# Autodesk Inventor assembly: Test Assembly
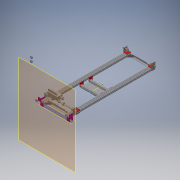
[picture p0: Inventor's stored thumbnail of the model, 180x180]
Saved by Autodesk Inventor 2016 SP2 (Build 200236200, 236)
## iProperties
Created: 2018-01-27
Part Number: Test Assembly
Document SubType Name: Assembly
Designer: CAD
Author: CAD
## Documents named in this file (20)
- C:\Users\CAD\Documents\GitHub\FIRST-ROBOTICS-2018-5436-CAD\Robot\Elevator\Test Assembly.iam
- C:\Users\CAD\Documents\GitHub\FIRST-ROBOTICS-2018-5436-CAD\Robot\Elevator\48 in 80-20 extrusion.ipt
- C:\Users\CAD\Documents\GitHub\FIRST-ROBOTICS-2018-5436-CAD\Robot\Elevator\80-20 extrusion rail.ipt
- C:\Users\CAD\Documents\GitHub\FIRST-ROBOTICS-2018-5436-CAD\Robot\Elevator\Bottom Elevator Bracket.ipt
- C:\Users\CAD\Documents\GitHub\FIRST-ROBOTICS-2018-5436-CAD\Robot\Elevator\10.75 in 80-20 extrusion.ipt
- C:\Users\CAD\Documents\GitHub\FIRST-ROBOTICS-2018-5436-CAD\Robot\Elevator\Triangle Bracket.ipt
- C:\Users\CAD\Documents\GitHub\FIRST-ROBOTICS-2018-5436-CAD\Robot\Elevator\11.25 in L.ipt
- C:\Users\CAD\Documents\GitHub\FIRST-ROBOTICS-2018-5436-CAD\Robot\Elevator\Upper Bracket of Elevator.ipt
- C:\Users\CAD\Documents\GitHub\FIRST-ROBOTICS-2018-5436-CAD\Robot\Elevator\hex axle for elevator.ipt
- C:\Users\CAD\Documents\GitHub\FIRST-ROBOTICS-2018-5436-CAD\Robot\Climbing Pieces\drive motor + trasmission pieces\Collar.ipt
- C:\Users\CAD\Documents\GitHub\FIRST-ROBOTICS-2018-5436-CAD\Robot\Elevator\Back Plate.ipt
- C:\Users\CAD\Documents\GitHub\FIRST-ROBOTICS-2018-5436-CAD\Robot\Elevator\Bearing.ipt
- C:\Users\CAD\Documents\GitHub\FIRST-ROBOTICS-2018-5436-CAD\Robot\Elevator\rope connection to cart.ipt
- C:\Users\CAD\Documents\GitHub\FIRST-ROBOTICS-2018-5436-CAD\Robot\Elevator\small hex axle top elevator.ipt
- C:\Users\CAD\Documents\GitHub\FIRST-ROBOTICS-2018-5436-CAD\Robot\Elevator\Bottom Elevator Bracket Square.ipt
- C:\Users\CAD\Documents\Vault\climbing\Climbing sprocket.ipt
- C:\Users\CAD\Documents\GitHub\FIRST-ROBOTICS-2018-5436-CAD\Robot\Elevator\Bag elevator Motor.ipt
- C:\Users\CAD\Documents\GitHub\FIRST-ROBOTICS-2018-5436-CAD\Robot\Elevator\Ls in motor tensioner.ipt
- C:\Users\CAD\Documents\GitHub\FIRST-ROBOTICS-2018-5436-CAD\Robot\Elevator\Motor Tension Block Mount.ipt
- C:\Users\CAD\Documents\GitHub\FIRST-ROBOTICS-2018-5436-CAD\Robot\Elevator\.5 in spacer.ipt
## Components (60 placed, 19 different names)
1. 48 in 80-20 extrusion:1 — Flush:1, Flush:3, Flush:5, Mate:16, Flush:12, Mate:26, Mate:27, Mate:70, Mate:71, Flush:27, Mate:83, Mate:84, Mate:98
2. 48 in 80-20 extrusion:2 — Flush:1, Mate:2, Mate:3, Mate:4, Mate:5, Flush:2, Mate:8, Mate:9, Mate:10, Mate:11, Flush:8, Flush:11, Mate:34, Mate:35, Mate:44, Mate:45, Mate:50, Mate:51, Mate:52, Mate:61, Mate:62, Flush:21
3. 48 in 80-20 extrusion:3 — Flush:5, Flush:6, Mate:19, Flush:11, Flush:13, Flush:14, Mate:39, Mate:40, Mate:46, Mate:47, Mate:53, Mate:54, Mate:58, Mate:59, Mate:60, Mate:67
4. 48 in 80-20 extrusion:4 — Flush:6, Mate:17, Mate:18, Mate:20, Mate:21, Flush:9, Flush:10, Flush:12, Mate:22, Mate:23, Mate:24, Mate:25, Mate:28, Mate:29, Flush:16, Mate:68, Mate:69, Mate:81, Mate:82, Flush:29, Mate:96
5. 80-20 extrusion rail:1 — Mate:2, Mate:3, Flush:2, Mate:6
6. 80-20 extrusion rail:2 — Mate:8, Mate:9, Flush:7, Mate:16
7. 80-20 extrusion rail:3 — Mate:10, Mate:11, Flush:8
8. 80-20 extrusion rail:4 — Mate:4, Mate:5, Flush:3, Mate:6, Flush:7
9. 80-20 extrusion rail:5 — Mate:17, Mate:18, Mate:19, Flush:9
10. 80-20 extrusion rail:8 — Mate:20, Mate:21, Flush:10
11. 80-20 extrusion rail:9 — Mate:24, Mate:25, Flush:14
12. 80-20 extrusion rail:10 — Mate:22, Mate:23, Flush:13
13. Bottom Elevator Bracket:1 — Mate:26, Mate:27, Flush:15, Angle:3, Flush:34, Mate:99
14. Bottom Elevator Bracket:2 — Mate:28, Mate:29, Flush:15, Flush:16, Mate:38, Flush:33, Mate:97, Flush:119
15. 80-20 extrusion rail:11 — Angle:2, Mate:39, Mate:40, Flush:17, Mate:41, Angle:4
16. 80-20 extrusion rail:12 — Mate:34, Mate:35, Angle:2, Flush:17, Mate:42, Mate:43, Mate:65
17. 10.75 in 80-20 extrusion:1 — Mate:41, Mate:42, Mate:43, Angle:4, Mate:66
18. Triangle Bracket:1 — Mate:44, Mate:45, Flush:18
19. Triangle Bracket:2 — Mate:46, Mate:47, Flush:18, Mate:48, Mate:49, Mate:67
20. 11.25 in L:1 — Mate:48, Mate:49, Mate:50
21. Triangle Bracket:3 — Mate:51, Mate:52, Mate:57, Flush:21
22. Triangle Bracket:4 — Mate:53, Mate:54, Mate:55, Mate:56
23. 11.25 in L:2 — Mate:55, Mate:56, Mate:57, Mate:58, Mate:65
24. 10.75 in 80-20 extrusion:2 — Mate:63, Mate:64, Angle:5, Mate:66, Mate:79, Flush:28, Mate:94, Mate:95
25. 80-20 extrusion rail:13 — Mate:59, Mate:60, Flush:19, Mate:63, Mate:80
26. 80-20 extrusion rail:14 — Mate:61, Mate:62, Flush:19, Mate:64, Angle:5
27. Upper Bracket of Elevator:1 — Mate:70, Mate:71, Flush:27, Insert:1
28. Upper Bracket of Elevator:2 — Mate:68, Mate:69, Mate:77, Flush:30, Insert:3, Mate:100
29. Collar:1 — Mate:73, Mate:74, Mate:77, Mate:87
30. Collar:2 — Mate:75, Mate:76, Mate:88
31. hex axle for elevator:1 — Mate:73, Mate:74, Mate:75, Mate:76, Flush:31, Mate:89, Mate:90, Mate:91, Mate:92, Mate:101, Mate:102, Mate:111, Mate:130, Mate:133, Mate:136
32. Back Plate:1 — Mate:79, Flush:28, Mate:80, Flush:32
33. Upper Bracket of Elevator:3 — Mate:83, Mate:84, Flush:30, Mate:85, Mate:86
34. Upper Bracket of Elevator:4 — Mate:81, Mate:82, Flush:29, Insert:2
35. Bearing:1 — Mate:85, Mate:86, Mate:87, Flush:31
36. Bearing:2 — Insert:2, Mate:109, Mate:138
37. Bearing:3 — Insert:3, Mate:88
38. Bearing:4 — Insert:1, Mate:106, Mate:137
39. rope connection to cart:1 — Mate:94, Mate:95, Flush:32
40. Collar:3 — Mate:89, Mate:90, Mate:93, Mate:103
41. Collar:4 — Mate:91, Mate:92, Mate:93
42. small hex axle top elevator:1 — Mate:108, Mate:135, Flush:128
43. small hex axle top elevator:2 — Mate:105, Mate:132, Flush:127
44. Bottom Elevator Bracket Square:1 — Flush:33, Mate:96, Mate:97, Mate:100
45. Bottom Elevator Bracket Square:3 — Mate:98, Flush:34, Mate:99
46. Climbing sprocket:1 — Mate:101, Mate:102, Mate:103, Mate:128
47. Climbing sprocket:2 — Mate:108, Mate:109, Mate:135, Flush:126, Mate:138, Flush:128
48. Climbing sprocket:3
49. Climbing sprocket:4 — Mate:130, Flush:126, Mate:136
50. Climbing sprocket:5 — Mate:105, Mate:106, Flush:35, Mate:132, Mate:137, Flush:127
51. Climbing sprocket:6 — Mate:111, Flush:35, Mate:133
52. Climbing sprocket:7 — Mate:120, Mate:121, Mate:122, Mate:123, Mate:124, Mate:128
53. Bag elevator Motor:1 — Mate:113, Flush:38, Flush:39, Mate:120, Mate:121, Mate:122, Mate:125, Mate:126
54. Ls in motor tensioner:1 — Mate:117, Flush:40, Flush:41, Flush:120
55. Ls in motor tensioner:2 — Mate:114, Mate:115, Mate:116, Mate:117, Flush:40, Flush:41
56. Motor Tension Block Mount:1 — Mate:113, Flush:38, Flush:39, Mate:114, Mate:115, Mate:116
57. .5 in spacer:1 — Mate:123, Mate:124, Mate:127
58. Collar:5 — Mate:125, Mate:126, Mate:127
59. Collar:6
60. Collar:7
## Relationships (159: Mate 115, Flush 37, Angle 4, Insert 3)
- Flush:1: 48 in 80-20 extrusion:1 ↔ 48 in 80-20 extrusion:2
- Mate:2: 48 in 80-20 extrusion:2 ↔ 80-20 extrusion rail:1
- Mate:3: 48 in 80-20 extrusion:2 ↔ 80-20 extrusion rail:1
- Mate:4: 48 in 80-20 extrusion:2 ↔ 80-20 extrusion rail:4
- Mate:5: 48 in 80-20 extrusion:2 ↔ 80-20 extrusion rail:4
- Flush:2 (101.6 mm): 48 in 80-20 extrusion:2 ↔ 80-20 extrusion rail:1
- Flush:3: 48 in 80-20 extrusion:1 ↔ 80-20 extrusion rail:4
- Mate:6 (136.7282 mm): 80-20 extrusion rail:1 ↔ 80-20 extrusion rail:4
- Flush:5: 48 in 80-20 extrusion:1 ↔ 48 in 80-20 extrusion:3
- Flush:6: 48 in 80-20 extrusion:3 ↔ 48 in 80-20 extrusion:4
- Mate:8: 48 in 80-20 extrusion:2 ↔ 80-20 extrusion rail:2
- Mate:9: 48 in 80-20 extrusion:2 ↔ 80-20 extrusion rail:2
- Flush:7: 80-20 extrusion rail:2 ↔ 80-20 extrusion rail:4
- Mate:10: 48 in 80-20 extrusion:2 ↔ 80-20 extrusion rail:3
- Mate:11: 48 in 80-20 extrusion:2 ↔ 80-20 extrusion rail:3
- Flush:8 (101.6 mm): 48 in 80-20 extrusion:2 ↔ 80-20 extrusion rail:3
- Mate:16: 48 in 80-20 extrusion:1 ↔ 80-20 extrusion rail:2
- Mate:17: 48 in 80-20 extrusion:4 ↔ 80-20 extrusion rail:5
- Mate:18: 48 in 80-20 extrusion:4 ↔ 80-20 extrusion rail:5
- Mate:19: 48 in 80-20 extrusion:3 ↔ 80-20 extrusion rail:5
- Mate:20: 48 in 80-20 extrusion:4 ↔ 80-20 extrusion rail:8
- Mate:21: 48 in 80-20 extrusion:4 ↔ 80-20 extrusion rail:8
- Flush:9: 48 in 80-20 extrusion:4 ↔ 80-20 extrusion rail:5
- Flush:10: 48 in 80-20 extrusion:4 ↔ 80-20 extrusion rail:8
- Flush:11: 48 in 80-20 extrusion:2 ↔ 48 in 80-20 extrusion:3
- Flush:12: 48 in 80-20 extrusion:1 ↔ 48 in 80-20 extrusion:4
- Mate:22: 48 in 80-20 extrusion:4 ↔ 80-20 extrusion rail:10
- Mate:23: 48 in 80-20 extrusion:4 ↔ 80-20 extrusion rail:10
- Flush:13 (101.6 mm): 48 in 80-20 extrusion:3 ↔ 80-20 extrusion rail:10
- Mate:24: 48 in 80-20 extrusion:4 ↔ 80-20 extrusion rail:9
- Mate:25: 48 in 80-20 extrusion:4 ↔ 80-20 extrusion rail:9
- Flush:14 (-101.6 mm): 48 in 80-20 extrusion:3 ↔ 80-20 extrusion rail:9
- Mate:26: 48 in 80-20 extrusion:1 ↔ Bottom Elevator Bracket:1
- Mate:27: 48 in 80-20 extrusion:1 ↔ Bottom Elevator Bracket:1
- Mate:28: 48 in 80-20 extrusion:4 ↔ Bottom Elevator Bracket:2
- Mate:29: 48 in 80-20 extrusion:4 ↔ Bottom Elevator Bracket:2
- Flush:15: Bottom Elevator Bracket:1 ↔ Bottom Elevator Bracket:2
- Flush:16: 48 in 80-20 extrusion:4 ↔ Bottom Elevator Bracket:2
- Mate:34: 48 in 80-20 extrusion:2 ↔ 80-20 extrusion rail:12
- Mate:35: 48 in 80-20 extrusion:2 ↔ 80-20 extrusion rail:12
- Angle:2 (0 deg): 80-20 extrusion rail:11 ↔ 80-20 extrusion rail:12
- Mate:38: Bottom Elevator Bracket:2
- Angle:3 (0 deg): Bottom Elevator Bracket:1
- Mate:39: 48 in 80-20 extrusion:3 ↔ 80-20 extrusion rail:11
- Mate:40: 48 in 80-20 extrusion:3 ↔ 80-20 extrusion rail:11
- Flush:17: 80-20 extrusion rail:11 ↔ 80-20 extrusion rail:12
- Mate:41: 80-20 extrusion rail:11 ↔ 10.75 in 80-20 extrusion:1
- Mate:42: 80-20 extrusion rail:12 ↔ 10.75 in 80-20 extrusion:1
- Mate:43: 80-20 extrusion rail:12 ↔ 10.75 in 80-20 extrusion:1
- Angle:4 (0 deg): 80-20 extrusion rail:11 ↔ 10.75 in 80-20 extrusion:1
- Mate:44: 48 in 80-20 extrusion:2 ↔ Triangle Bracket:1
- Mate:45: 48 in 80-20 extrusion:2 ↔ Triangle Bracket:1
- Mate:46: 48 in 80-20 extrusion:3 ↔ Triangle Bracket:2
- Mate:47: 48 in 80-20 extrusion:3 ↔ Triangle Bracket:2
- Flush:18: Triangle Bracket:1 ↔ Triangle Bracket:2
- Mate:48: Triangle Bracket:2 ↔ 11.25 in L:1
- Mate:49: Triangle Bracket:2 ↔ 11.25 in L:1
- Mate:50 (1.27 mm): 48 in 80-20 extrusion:2 ↔ 11.25 in L:1
- Mate:51: 48 in 80-20 extrusion:2 ↔ Triangle Bracket:3
- Mate:52: 48 in 80-20 extrusion:2 ↔ Triangle Bracket:3
- Mate:53: 48 in 80-20 extrusion:3 ↔ Triangle Bracket:4
- Mate:54: 48 in 80-20 extrusion:3 ↔ Triangle Bracket:4
- Mate:55: Triangle Bracket:4 ↔ 11.25 in L:2
- Mate:56: Triangle Bracket:4 ↔ 11.25 in L:2
- Mate:57: Triangle Bracket:3 ↔ 11.25 in L:2
- Mate:58 (1.27 mm): 48 in 80-20 extrusion:3 ↔ 11.25 in L:2
- Mate:59: 48 in 80-20 extrusion:3 ↔ 80-20 extrusion rail:13
- Mate:60: 48 in 80-20 extrusion:3 ↔ 80-20 extrusion rail:13
- Mate:61: 48 in 80-20 extrusion:2 ↔ 80-20 extrusion rail:14
- Mate:62: 48 in 80-20 extrusion:2 ↔ 80-20 extrusion rail:14
- Flush:19: 80-20 extrusion rail:13 ↔ 80-20 extrusion rail:14
- Mate:63: 10.75 in 80-20 extrusion:2 ↔ 80-20 extrusion rail:13
- Mate:64: 10.75 in 80-20 extrusion:2 ↔ 80-20 extrusion rail:14
- Flush:21: 48 in 80-20 extrusion:2 ↔ Triangle Bracket:3
- Mate:65: 80-20 extrusion rail:12 ↔ 11.25 in L:2
- Angle:5 (0 deg): 10.75 in 80-20 extrusion:2 ↔ 80-20 extrusion rail:14
- Mate:66 (101.6 mm): 10.75 in 80-20 extrusion:1 ↔ 10.75 in 80-20 extrusion:2
- Mate:67 (-60.325 mm): 48 in 80-20 extrusion:3 ↔ Triangle Bracket:2
- Mate:68: 48 in 80-20 extrusion:4 ↔ Upper Bracket of Elevator:2
- Mate:69: 48 in 80-20 extrusion:4 ↔ Upper Bracket of Elevator:2
- Mate:70: 48 in 80-20 extrusion:1 ↔ Upper Bracket of Elevator:1
- Mate:71: 48 in 80-20 extrusion:1 ↔ Upper Bracket of Elevator:1
- Mate:73: Collar:1 ↔ hex axle for elevator:1
- Mate:74: Collar:1 ↔ hex axle for elevator:1
- Mate:75: Collar:2 ↔ hex axle for elevator:1
- Mate:76: Collar:2 ↔ hex axle for elevator:1
- Mate:77: Upper Bracket of Elevator:2 ↔ Collar:1
- Flush:27: 48 in 80-20 extrusion:1 ↔ Upper Bracket of Elevator:1
- Mate:79: 10.75 in 80-20 extrusion:2 ↔ Back Plate:1
- Flush:28: 10.75 in 80-20 extrusion:2 ↔ Back Plate:1
- Mate:80: 80-20 extrusion rail:13 ↔ Back Plate:1
- Mate:81: 48 in 80-20 extrusion:4 ↔ Upper Bracket of Elevator:4
- Mate:82: 48 in 80-20 extrusion:4 ↔ Upper Bracket of Elevator:4
- Flush:29: 48 in 80-20 extrusion:4 ↔ Upper Bracket of Elevator:4
- Mate:83: 48 in 80-20 extrusion:1 ↔ Upper Bracket of Elevator:3
- Mate:84: 48 in 80-20 extrusion:1 ↔ Upper Bracket of Elevator:3
- Flush:30: Upper Bracket of Elevator:2 ↔ Upper Bracket of Elevator:3
- Mate:85: Upper Bracket of Elevator:3 ↔ Bearing:1
- Mate:86: Upper Bracket of Elevator:3 ↔ Bearing:1
- Insert:1: Upper Bracket of Elevator:1 ↔ Bearing:4
- Insert:2: Upper Bracket of Elevator:4 ↔ Bearing:2
- Insert:3: Upper Bracket of Elevator:2 ↔ Bearing:3
- Mate:87: Collar:1 ↔ Bearing:1
- Mate:88: Collar:2 ↔ Bearing:3
- Flush:31 (-23.5585 mm): hex axle for elevator:1 ↔ Bearing:1
- Mate:89: hex axle for elevator:1 ↔ Collar:3
- Mate:90: hex axle for elevator:1 ↔ Collar:3
- Mate:91: hex axle for elevator:1 ↔ Collar:4
- Mate:92: hex axle for elevator:1 ↔ Collar:4
- Mate:93 (50.8 mm): Collar:3 ↔ Collar:4
- Mate:94: 10.75 in 80-20 extrusion:2 ↔ rope connection to cart:1
- Mate:95: 10.75 in 80-20 extrusion:2 ↔ rope connection to cart:1
- Flush:32: Back Plate:1 ↔ rope connection to cart:1
- Flush:33: Bottom Elevator Bracket:2 ↔ Bottom Elevator Bracket Square:1
- Mate:96: 48 in 80-20 extrusion:4 ↔ Bottom Elevator Bracket Square:1
- Mate:97: Bottom Elevator Bracket:2 ↔ Bottom Elevator Bracket Square:1
- Mate:98: 48 in 80-20 extrusion:1 ↔ Bottom Elevator Bracket Square:3
- Flush:34: Bottom Elevator Bracket:1 ↔ Bottom Elevator Bracket Square:3
- Mate:99: Bottom Elevator Bracket:1 ↔ Bottom Elevator Bracket Square:3
- Mate:100: Upper Bracket of Elevator:2 ↔ Bottom Elevator Bracket Square:1
- Mate:101: hex axle for elevator:1 ↔ Climbing sprocket:1
- Mate:102: hex axle for elevator:1 ↔ Climbing sprocket:1
- Mate:103: Collar:3 ↔ Climbing sprocket:1
- Mate:105: small hex axle top elevator:2 ↔ Climbing sprocket:5
- Mate:106: Bearing:4 ↔ Climbing sprocket:5
- Mate:108: small hex axle top elevator:1 ↔ Climbing sprocket:2
- Mate:109: Bearing:2 ↔ Climbing sprocket:2
- Mate:111: hex axle for elevator:1 ↔ Climbing sprocket:6
- Flush:35: Climbing sprocket:5 ↔ Climbing sprocket:6
- Mate:113: Bag elevator Motor:1 ↔ Motor Tension Block Mount:1
- Flush:38: Bag elevator Motor:1 ↔ Motor Tension Block Mount:1
- Flush:39 (3.175 mm): Bag elevator Motor:1 ↔ Motor Tension Block Mount:1
- Mate:114: Ls in motor tensioner:2 ↔ Motor Tension Block Mount:1
- Mate:115: Ls in motor tensioner:2 ↔ Motor Tension Block Mount:1
- Mate:116: Ls in motor tensioner:2 ↔ Motor Tension Block Mount:1
- Mate:117 (114.3 mm): Ls in motor tensioner:1 ↔ Ls in motor tensioner:2
- Flush:40: Ls in motor tensioner:1 ↔ Ls in motor tensioner:2
- Flush:41: Ls in motor tensioner:1 ↔ Ls in motor tensioner:2
- Flush:119: Bottom Elevator Bracket:2
- Flush:120: Ls in motor tensioner:1
- Mate:120: Climbing sprocket:7 ↔ Bag elevator Motor:1
- Mate:121: Climbing sprocket:7 ↔ Bag elevator Motor:1
- Mate:122 (2.54 mm): Climbing sprocket:7 ↔ Bag elevator Motor:1
- Mate:123: Climbing sprocket:7 ↔ .5 in spacer:1
- Mate:124: Climbing sprocket:7 ↔ .5 in spacer:1
- Mate:125: Bag elevator Motor:1 ↔ Collar:5
- Mate:126: Bag elevator Motor:1 ↔ Collar:5
- Mate:127: .5 in spacer:1 ↔ Collar:5
- Mate:128: Climbing sprocket:1 ↔ Climbing sprocket:7
- Mate:130: hex axle for elevator:1 ↔ Climbing sprocket:4
- Mate:132: small hex axle top elevator:2 ↔ Climbing sprocket:5
- Mate:133: hex axle for elevator:1 ↔ Climbing sprocket:6
- Mate:135: small hex axle top elevator:1 ↔ Climbing sprocket:2
- Flush:126: Climbing sprocket:2 ↔ Climbing sprocket:4
- Mate:136: hex axle for elevator:1 ↔ Climbing sprocket:4
- Mate:137 (22.225 mm): Bearing:4 ↔ Climbing sprocket:5
- Flush:127 (-12.7 mm): small hex axle top elevator:2 ↔ Climbing sprocket:5
- Mate:138 (22.225 mm): Bearing:2 ↔ Climbing sprocket:2
- Flush:128 (12.7 mm): small hex axle top elevator:1 ↔ Climbing sprocket:2
